# Autodesk Inventor assembly: skeleton
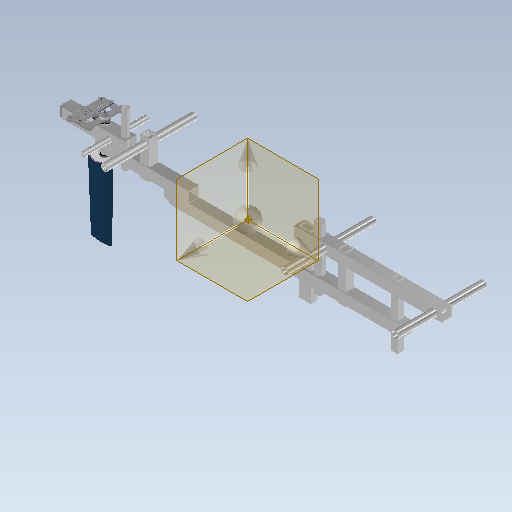
[picture p0: Inventor's stored thumbnail of the model, 512x512]
Saved by Autodesk Inventor 2020 (Build 240168000, 168)
## iProperties
Created: 2016-11-14
Part Number: skeleton
Document SubType Name: Assembly
Designer: jous
Mass: 1497.72 g
Surface Area: 11859.7 cm^2
Volume: 1497.72 cm^3
Density: 1 g/cm^3
Author: jous
## Documents named in this file (12)
- C:\Users\jous\Desktop\boat\skeleton.iam
- C:\Users\jous\Desktop\boat\skeleton.ipt
- C:\Users\jous\Desktop\boat\rudder_horn.ipt
- C:\Users\jous\Desktop\boat\H4FM_0405_04.ipt
- C:\Users\jous\Desktop\boat\rudder_acryl_ring.ipt
- C:\Users\jous\Desktop\boat\rudder_polycarb_seal.ipt
- C:\Users\jous\Desktop\boat\seal.ipt
- C:\Users\jous\Desktop\boat\rudder_printed_bushing.ipt
- C:\Users\jous\Desktop\boat\H1FI-0809-16.ipt
- C:\Users\jous\Desktop\boat\washer6.ipt
- C:\Users\jous\Desktop\boat\rudder.ipt
- C:\Users\jous\Desktop\boat\motor_assembly.iam
## Components (16 placed, 11 different names)
1. skeleton:1 — Rotational:20, Rotational:21, Mate:1, Rotational:29
2. rudder_horn:1 — Rotational:25, Rotational:26, Rotational:27
3. H4FM_0405_04:1 — Rotational:27
4. H4FM_0405_04:2 — Rotational:26
5. rudder_acryl_ring:1 — Rigid:1, Rotational:21
6. rudder_polycarb_seal:1 — Rigid:1, Rotational:14
7. seal:1 — Rotational:14, Rotational:15
8. seal:2 — Rotational:15
9. rudder_printed_bushing:1 — Rotational:17, Rotational:29
10. H1FI-0809-16:1 — Rotational:17, Rotational:23
11. rudder_printed_bushing:2 — Rotational:19, Rotational:20
12. H1FI-0809-16:2 — Rotational:19, Rotational:22
13. washer6:1 — Rotational:22, Rotational:25
14. washer6:2 — Rotational:23, Rotational:30
15. rudder:1 — Rotational:30
16. motor_assembly:1 [sub-assembly] — Mate:1
## Relationships (15: RevoluteJoint 13, WeldJoint 1, Mate 1)
- Rigid:1 [WeldJoint]: rudder_acryl_ring:1 ↔ rudder_polycarb_seal:1
- Rotational:14 [RevoluteJoint]: rudder_polycarb_seal:1 ↔ seal:1
- Rotational:15 [RevoluteJoint]: seal:1 ↔ seal:2
- Rotational:17 [RevoluteJoint]: rudder_printed_bushing:1 ↔ H1FI-0809-16:1
- Rotational:19 [RevoluteJoint]: rudder_printed_bushing:2 ↔ H1FI-0809-16:2
- Rotational:20 [RevoluteJoint]: skeleton:1 ↔ rudder_printed_bushing:2
- Rotational:21 [RevoluteJoint] (30 mm): skeleton:1 ↔ rudder_acryl_ring:1
- Rotational:22 [RevoluteJoint]: H1FI-0809-16:2 ↔ washer6:1
- Rotational:23 [RevoluteJoint]: H1FI-0809-16:1 ↔ washer6:2
- Rotational:25 [RevoluteJoint]: rudder_horn:1 ↔ washer6:1
- Mate:1: skeleton:1 ↔ motor_assembly:1
- Rotational:26 [RevoluteJoint]: rudder_horn:1 ↔ H4FM_0405_04:2
- Rotational:27 [RevoluteJoint]: rudder_horn:1 ↔ H4FM_0405_04:1
- Rotational:29 [RevoluteJoint]: skeleton:1 ↔ rudder_printed_bushing:1
- Rotational:30 [RevoluteJoint]: washer6:2 ↔ rudder:1
